# Autodesk Inventor assembly: Assembly1
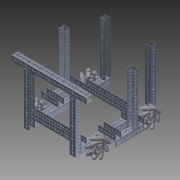
[picture p0: Inventor's stored thumbnail of the model, 180x180]
Saved by Autodesk Inventor 2015 (Build 190159000, 159)
## iProperties
Created: 2014-11-05
Part Number: Assembly1
Document SubType Name: Assembly
Designer: Evan
Author: Evan
## Documents named in this file (7)
- C:\Users\Evan\Desktop\Cad ftc robot\New folder\Assembly1.iam
- C:\Users\Evan\Desktop\Cad ftc robot\New folder\robot.iam
- C:\Users\Evan\Desktop\Cad ftc robot\New folder\robot_MIR.iam
- C:\Users\Evan\Desktop\Cad ftc robot\New folder\Official Tetrix Parts .STEP\Official Tetrix Parts .step\Tetrix_Kit - Ring_it_up\Tetrix_Kit_FTC\Imported Components\tetrix_739068_2012_288_channel\tetrix_739068_201.ipt
- C:\Users\Evan\Desktop\Cad ftc robot\New folder\Official Tetrix Parts .STEP\Official Tetrix Parts .step\Tetrix_Kit - Ring_it_up\Tetrix_Kit_FTC\Imported Components\tetrix_739062_2012\tetrix_739062_2012.ipt
- C:\Users\Evan\Desktop\Cad ftc robot\New folder\Official Tetrix Parts .STEP\Official Tetrix Parts .step\Tetrix_Kit - Ring_it_up\Tetrix_Kit_FTC\Imported Components\tetrix_739069_2012_416_channel\tetrix_739069_201.ipt
- C:\Users\Evan\Desktop\Cad ftc robot\New folder\Official Tetrix Parts .STEP\Official Tetrix Parts .step\Tetrix_Kit - Ring_it_up\Tetrix_Kit_FTC\Imported Components\tetrix_739065_2012_32_channel\tetrix_739065_2012.ipt
## Components (15 placed, 6 different names)
1. robot:1 [sub-assembly] — Mate:2, Mate:3, Mate:6, Mate:16
2. robot_MIR:1 [sub-assembly] — Mate:1, Mate:7, Mate:15
3. tetrix_739068_201:1 — Mate:1, Mate:2, Mate:4, Mate:5
4. tetrix_739068_201:2 — Mate:9
5. tetrix_739068_201:3 — Mate:5, Mate:10
6. tetrix_739068_201:4 — Mate:4, Mate:11
7. tetrix_739068_201:5 — Mate:8
8. tetrix_739068_201:6 — Mate:3
9. tetrix_739062_2012:1 — Mate:7, Mate:8
10. tetrix_739062_2012:2 — Mate:6, Mate:9
11. tetrix_739065_2012:1 — Mate:11, Mate:14
12. tetrix_739065_2012:2 — Mate:10
13. tetrix_739069_201:3 — Mate:14
14. tetrix_739068_201:7 — Mate:16
15. tetrix_739068_201:8 — Mate:15
## Relationships (14: Mate 14)
- Mate:1: robot_MIR:1 ↔ tetrix_739068_201:1
- Mate:2: robot:1 ↔ tetrix_739068_201:1
- Mate:3: robot:1 ↔ tetrix_739068_201:6
- Mate:4: tetrix_739068_201:1 ↔ tetrix_739068_201:4
- Mate:5: tetrix_739068_201:1 ↔ tetrix_739068_201:3
- Mate:6: robot:1 ↔ tetrix_739062_2012:2
- Mate:7: robot_MIR:1 ↔ tetrix_739062_2012:1
- Mate:8: tetrix_739068_201:5 ↔ tetrix_739062_2012:1
- Mate:9: tetrix_739068_201:2 ↔ tetrix_739062_2012:2
- Mate:10: tetrix_739068_201:3 ↔ tetrix_739065_2012:2
- Mate:11: tetrix_739068_201:4 ↔ tetrix_739065_2012:1
- Mate:14: tetrix_739065_2012:1 ↔ tetrix_739069_201:3
- Mate:15: robot_MIR:1 ↔ tetrix_739068_201:8
- Mate:16: robot:1 ↔ tetrix_739068_201:7
